# Autodesk Inventor assembly: servo_metallic_600TVL
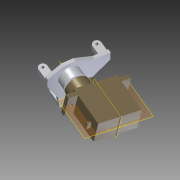
[picture p0: Inventor's stored thumbnail of the model, 180x180]
Saved by Autodesk Inventor 2015 SP1 (Build 190203100, 203)
## iProperties
Created: 2015-07-09
Part Number: servo_metallic_600TVL
Document SubType Name: Assembly
Designer: Alexandre Cherpillod
Author: Alexandre Cherpillod
## Documents named in this file (4)
- D:\_windows\_github_doc\MAVRIC\Mechanics\myCopter_CAD\Inventor\Gimbal_Servo\servo_FatShark_180MG.iam
- D:\_windows\_github_doc\MAVRIC\Mechanics\myCopter_CAD\Inventor\Gimbal_Servo\servo_FatShark_180MG.ipt
- D:\_windows\_github_doc\MAVRIC\Mechanics\myCopter_CAD\Inventor\Gimbal_Servo\shaft_nut_for_FatShark_180MG.ipt
- D:\_windows\_github_doc\MAVRIC\Mechanics\myCopter_CAD\Inventor\Gimbal_Servo\servo_gimbal_interpart_1.ipt
## Components (3 placed, 3 different names)
1. servo_FatShark_180MG:1 — Mate:1, Flush:1
2. shaft_nut_for_FatShark_180MG:1 — Mate:1, Flush:1, Mate:2, Mate:3, Mate:4
3. servo_gimbal_interpart_1:1 — Mate:2, Mate:3, Mate:4
## Relationships (5: Mate 4, Flush 1)
- Mate:1: servo_FatShark_180MG:1 ↔ shaft_nut_for_FatShark_180MG:1
- Flush:1 (-5 mm): servo_FatShark_180MG:1 ↔ shaft_nut_for_FatShark_180MG:1
- Mate:2: shaft_nut_for_FatShark_180MG:1 ↔ servo_gimbal_interpart_1:1
- Mate:3: shaft_nut_for_FatShark_180MG:1 ↔ servo_gimbal_interpart_1:1
- Mate:4: shaft_nut_for_FatShark_180MG:1 ↔ servo_gimbal_interpart_1:1
